# Autodesk Inventor assembly: ForearmLeft
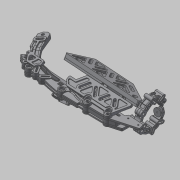
[picture p0: Inventor's stored thumbnail of the model, 180x180]
Saved by Autodesk Inventor 2015 SP1 (Build 190203100, 203)
## iProperties
Created: 2016-10-02
Part Number: ForearmLeft
Document SubType Name: Assembly
Designer: Val
Author: Val
## Documents named in this file (16)
- C:\Users\Val\Desktop\ExoGit\elysium-max-exoskeleton\src\Assemblies\ForearmRight.iam
- C:\Users\Val\Desktop\ExoGit\elysium-max-exoskeleton\src\ForearmInnerBase.ipt
- C:\Users\Val\Desktop\ExoGit\elysium-max-exoskeleton\src\ForearmPistonConnector.ipt
- C:\Users\Val\Desktop\ExoGit\elysium-max-exoskeleton\src\ForearmClamp.ipt
- C:\Users\Val\Desktop\ExoGit\elysium-max-exoskeleton\src\ForearmClampHead.ipt
- C:\Users\Val\Desktop\ExoGit\elysium-max-exoskeleton\src\ForearmClampLink.ipt
- C:\Users\Val\Desktop\ExoGit\elysium-max-exoskeleton\src\ForearmCuffConnector.ipt
- C:\Users\Val\Desktop\ExoGit\elysium-max-exoskeleton\src\ForearmBase.ipt
- C:\Users\Val\Desktop\ExoGit\elysium-max-exoskeleton\src\ForearmLowerShockPlateRight.ipt
- C:\Users\Val\Desktop\ExoGit\elysium-max-exoskeleton\src\ForearmUpperShockPlateRight.ipt
- C:\Users\Val\Desktop\ExoGit\elysium-max-exoskeleton\src\UpperForearmRight.ipt
- C:\Users\Val\Desktop\ExoGit\elysium-max-exoskeleton\src\UpperForearmShockPlateConnectorRight.ipt
- C:\Users\Val\Desktop\ExoGit\elysium-max-exoskeleton\src\LowerForearm.ipt
- C:\Users\Val\Desktop\ExoGit\elysium-max-exoskeleton\src\ElbowConnectorLinkRight.ipt
- C:\Users\Val\Desktop\ExoGit\elysium-max-exoskeleton\src\ElbowConnectorRight.ipt
- C:\Users\Val\Desktop\ExoGit\elysium-max-exoskeleton\src\ElbowConnectorUnderlinkRight.ipt
## Components (22 placed, 15 different names)
1. ForearmInnerBase:1 — Mate:36, Mate:37, Mate:38, Mate:58, Mate:59
2. ForearmPistonConnector:1
3. ForearmClamp:1 — Flush:29, Mate:28, Rotational:2
4. ForearmClamp:2 — Mate:29, Flush:30, Rotational:1
5. ForearmClampHead:1 — Flush:29, Mate:28
6. ForearmClampHead:2 — Mate:29, Flush:30
7. ForearmClampLink:1 — Rotational:1, Rotational:2, Rotational:3, Mate:35
8. ForearmCuffConnector:1 — Rotational:3, Mate:45, Mate:47
9. ForearmCuffConnector:2 — Mate:35, Mate:46, Mate:48
10. ForearmPistonConnector:2
11. ForearmPistonConnector:3
12. ForearmPistonConnector:4
13. ForearmPistonConnector:5
14. ForearmBase:1 — Mate:36, Mate:37, Mate:38, Mate:39, Mate:40, Mate:41
15. ForearmLowerShockPlateRight:1 — Mate:52, Mate:53, Mate:54
16. ForearmUpperShockPlateRight:1 — Mate:55, Mate:56, Mate:57
17. UpperForearmRight:1 — Mate:39, Mate:40, Mate:41, Mate:42, Mate:43, Mate:44, Mate:51
18. UpperForearmShockPlateConnectorRight:1 — Mate:49, Mate:50, Mate:51, Mate:55, Mate:56, Mate:57
19. LowerForearm:1 — Mate:42, Mate:43, Mate:44, Mate:45, Mate:46, Mate:47, Mate:48, Mate:49, Mate:50, Mate:52, Mate:53, Mate:54
20. ElbowConnectorLinkRight:1 — Mate:60, Mate:61, Angle:1, Mate:62, Mate:63, Mate:64
21. ElbowConnectorRight:1 — Mate:62, Mate:63, Mate:64
22. ElbowConnectorUnderlinkRight:1 — Mate:58, Mate:59, Mate:60, Mate:61, Angle:1
## Relationships (38: Mate 32, RevoluteJoint 3, Flush 2, Angle 1)
- Flush:29 (3 mm): ForearmClamp:1 ↔ ForearmClampHead:1
- Mate:28: ForearmClamp:1 ↔ ForearmClampHead:1
- Mate:29: ForearmClamp:2 ↔ ForearmClampHead:2
- Flush:30 (3 mm): ForearmClamp:2 ↔ ForearmClampHead:2
- Rotational:1 [RevoluteJoint]: ForearmClamp:2 ↔ ForearmClampLink:1
- Rotational:2 [RevoluteJoint]: ForearmClamp:1 ↔ ForearmClampLink:1
- Rotational:3 [RevoluteJoint]: ForearmClampLink:1 ↔ ForearmCuffConnector:1
- Mate:35: ForearmClampLink:1 ↔ ForearmCuffConnector:2
- Mate:36: ForearmInnerBase:1 ↔ ForearmBase:1
- Mate:37: ForearmInnerBase:1 ↔ ForearmBase:1
- Mate:38: ForearmInnerBase:1 ↔ ForearmBase:1
- Mate:39: ForearmBase:1 ↔ UpperForearmRight:1
- Mate:40: ForearmBase:1 ↔ UpperForearmRight:1
- Mate:41: ForearmBase:1 ↔ UpperForearmRight:1
- Mate:42: UpperForearmRight:1 ↔ LowerForearm:1
- Mate:43: UpperForearmRight:1 ↔ LowerForearm:1
- Mate:44: UpperForearmRight:1 ↔ LowerForearm:1
- Mate:45: ForearmCuffConnector:1 ↔ LowerForearm:1
- Mate:46: ForearmCuffConnector:2 ↔ LowerForearm:1
- Mate:47: ForearmCuffConnector:1 ↔ LowerForearm:1
- Mate:48: ForearmCuffConnector:2 ↔ LowerForearm:1
- Mate:49: UpperForearmShockPlateConnectorRight:1 ↔ LowerForearm:1
- Mate:50: UpperForearmShockPlateConnectorRight:1 ↔ LowerForearm:1
- Mate:51: UpperForearmRight:1 ↔ UpperForearmShockPlateConnectorRight:1
- Mate:52: ForearmLowerShockPlateRight:1 ↔ LowerForearm:1
- Mate:53: ForearmLowerShockPlateRight:1 ↔ LowerForearm:1
- Mate:54: ForearmLowerShockPlateRight:1 ↔ LowerForearm:1
- Mate:55: ForearmUpperShockPlateRight:1 ↔ UpperForearmShockPlateConnectorRight:1
- Mate:56: ForearmUpperShockPlateRight:1 ↔ UpperForearmShockPlateConnectorRight:1
- Mate:57: ForearmUpperShockPlateRight:1 ↔ UpperForearmShockPlateConnectorRight:1
- Mate:58: ForearmInnerBase:1 ↔ ElbowConnectorUnderlinkRight:1
- Mate:59: ForearmInnerBase:1 ↔ ElbowConnectorUnderlinkRight:1
- Mate:60: ElbowConnectorLinkRight:1 ↔ ElbowConnectorUnderlinkRight:1
- Mate:61: ElbowConnectorLinkRight:1 ↔ ElbowConnectorUnderlinkRight:1
- Angle:1 (0 deg): ElbowConnectorLinkRight:1 ↔ ElbowConnectorUnderlinkRight:1
- Mate:62: ElbowConnectorLinkRight:1 ↔ ElbowConnectorRight:1
- Mate:63: ElbowConnectorLinkRight:1 ↔ ElbowConnectorRight:1
- Mate:64: ElbowConnectorLinkRight:1 ↔ ElbowConnectorRight:1
